# Autodesk Inventor assembly: total
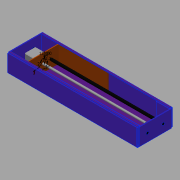
[picture p0: Inventor's stored thumbnail of the model, 180x180]
Saved by Autodesk Inventor 2016 (Build 200138000, 138)
## iProperties
Created: 2015-10-11
Part Number: total
Document SubType Name: Assembly
Designer: daniel
Author: daniel
## Documents named in this file (6)
- C:\Users\daniel\Documents\GitHub\cardboard-stage-metric\stage\total.iam
- C:\Users\daniel\Documents\GitHub\cardboard-stage-metric\stage\a.iam
- C:\Users\daniel\Documents\GitHub\cardboard-stage-metric\stage\carriage.iam
- C:\Users\daniel\Documents\GitHub\cardboard-stage-metric\stage\shaft.ipt
- C:\Users\daniel\Documents\GitHub\cardboard-stage-metric\stage\b1.iam
- C:\Users\daniel\Documents\GitHub\cardboard-stage-metric\stage\nema17.ipt
## Components (6 placed, 5 different names)
1. a:1 [sub-assembly] — Insert:1, Insert:2, Flush:1, Flush:2, Flush:3, Mate:1, Mate:2
2. carriage:1 [sub-assembly] — Cylindrical:1
3. shaft:1 — Insert:1
4. shaft:2 — Insert:2, Cylindrical:1
5. b1:1 [sub-assembly] — Mate:1, Mate:2, Insert:3
6. nema17:1 — Insert:3
## Relationships (9: Insert 3, Flush 3, Mate 2, CylindricalJoint 1)
- Insert:1: a:1 ↔ shaft:1
- Insert:2: a:1 ↔ shaft:2
- Cylindrical:1: carriage:1 ↔ shaft:2
- Flush:1: a:1
- Flush:2: a:1
- Flush:3: a:1
- Mate:1: a:1 ↔ b1:1
- Mate:2: a:1 ↔ b1:1
- Insert:3 (10 mm): b1:1 ↔ nema17:1
